# Autodesk Inventor assembly: 組合1
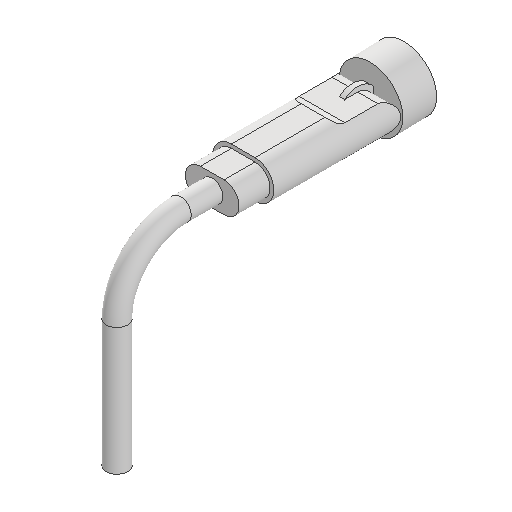
[picture p0: Inventor's stored thumbnail of the model, 512x512]
Saved by Autodesk Inventor 2025.2 (Build 292293000, 293)
## iProperties
Created: 2025-07-21
Part Number: 組合1
Document SubType Name: Assembly
Designer: jna1j
Author: jna1j
## Documents named in this file (3)
- G:\我的雲端硬碟\作業\113-2\燈燈燈燈\磁吸線\組合1.iam
- G:\我的雲端硬碟\作業\113-2\燈燈燈燈\磁吸線\萬向頭.ipt
- G:\我的雲端硬碟\作業\113-2\燈燈燈燈\磁吸線\基座.ipt
## Components (2 placed, 2 different names)
1. 萬向頭:1 — 貼合:1, 貼合:2
2. 基座:1 — 貼合:1, 貼合:2
## Relationships (2: Mate 2)
- 貼合:1 [Mate]: 萬向頭:1 ↔ 基座:1
- 貼合:2 [Mate]: 萬向頭:1 ↔ 基座:1
